# Autodesk Inventor assembly: 2AM-17-A-5200 - claw
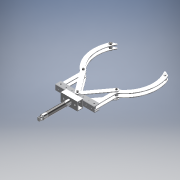
[picture p0: Inventor's stored thumbnail of the model, 180x180]
Saved by Autodesk Inventor 2017 (Build 210142000, 142)
## iProperties
Created: 2017-12-27
Part Number: 2AM-17-A-5200 - claw
Document SubType Name: Assembly
Designer: Micah
Mass: 406.083 g
Surface Area: 1172.05 cm^2
Volume: 145.474 cm^3
Density: 2.79145 g/cm^3
Author: Micah
## Documents named in this file (12)
- C:\Users\Micah\Desktop\inventor\CADathon-2017\2AM-17-A-0200 - Smokestack Elevator\2AM-17-A-5200 - claw.iam
- C:\Users\Micah\Desktop\inventor\CADathon-2017\2AM-17-A-0200 - Smokestack Elevator\2AM-17-A-6200 - claw arm.iam
- C:\Users\Micah\Desktop\inventor\CADathon-2017\2AM-17-A-0200 - Smokestack Elevator\2AM-17-P-5204 - links.ipt
- C:\Users\Micah\Desktop\inventor\CADathon-2017\2AM-17-A-0200 - Smokestack Elevator\2AM-17-P-5205 - c channel.ipt
- C:\Users\Micah\Desktop\inventor\CADathon-2017\2AM-17-A-0200 - Smokestack Elevator\2AM-17-P-5207 - supports spacer 09.ipt
- C:\Users\Micah\Desktop\inventor\CADathon-2017\2AM-17-A-0200 - Smokestack Elevator\2AM-17-P-5208 - supports spacer 215.ipt
- C:\Users\Micah\Desktop\inventor\CADathon-2017\2AM-17-A-0200 - Smokestack Elevator\2AM-17-P-5209 - cylinder mount.ipt
- C:\Users\Micah\Desktop\inventor\CADathon-2017\2AM-17-A-0200 - Smokestack Elevator\COTS\PARTserver02017093005073711525079192d056f\AIS2016\042-DP(F,D-166-3)(F,D-9).iam
- C:\Users\Micah\Documents\Inventor\Content Center Files\R2017\en-US\IS 2269\IS 2269 - M5 x 40.ipt
- C:\Users\Micah\Desktop\inventor\CADathon-2017\2AM-17-A-0200 - Smokestack Elevator\COTS\PARTserver02017093005073711525079192d056f\AIS2016\rod1.iam
- C:\Users\Micah\Documents\Inventor\Content Center Files\R2017\en-US\ISO 4762(2)\ISO 4762 - M5 x 45ISO.ipt
- C:\Users\Micah\Documents\Inventor\Content Center Files\R2017\en-US\ANSI B18.2.4.5M\ANSI B18.2.4.5M - M5 x 0.8.ipt
## Components (20 placed, 11 different names)
1. 2AM-17-A-6200 - claw arm:1 [sub-assembly] — Mate:9, Mate:11, Rotational:1, Rotational:4
2. 2AM-17-P-5204 - links:1 — Mate:3, Mate:13, Flush:1, Insert:1, Insert:5
3. 2AM-17-P-5204 - links:2 — Mate:4, Cylindrical:1, Mate:15, Flush:1, Mate:27
4. 2AM-17-P-5204 - links:4 — Mate:3, Cylindrical:2, Mate:14, Flush:2, Insert:2
5. 2AM-17-P-5205 - c channel:1 — Cylindrical:1, Cylindrical:2, Mate:9, Mate:10, Mate:11, Mate:16, Mate:17, Mate:18, Mate:19
6. 2AM-17-P-5204 - links:5 — Mate:4, Mate:12, Flush:2, Mate:23, Mate:25
7. 2AM-17-A-6200 - claw arm:2 [sub-assembly] — Mate:10, Mate:16, Rotational:2, Rotational:3
8. 2AM-17-P-5207 - supports spacer 09:1 — Mate:15, Rotational:2
9. 2AM-17-P-5207 - supports spacer 09:2 — Mate:14, Rotational:4
10. 2AM-17-P-5208 - supports spacer 215:1 — Mate:12, Rotational:1
11. 2AM-17-P-5208 - supports spacer 215:2 — Mate:13, Rotational:3
12. 2AM-17-P-5209 - cylinder mount:1 — Mate:17, Mate:18, Mate:19, Mate:20
13. 042-DP(F,D-166-3)(F,D-9):1 [sub-assembly] — Mate:20, Mate:21
14. rod1:1 [sub-assembly] — Mate:21
15. IS 2269 M5 x 40:1 — Insert:1, Mate:26
16. IS 2269 M5 x 40:2 — Insert:2, Mate:24
17. ISO 4762 M5 x 45:1 — Insert:5, Mate:22
18. Hex Jam Nut - Metric M5 x 0.8:1 — Mate:22, Mate:23
19. Hex Jam Nut - Metric M5 x 0.8:2 — Mate:24, Mate:25
20. Hex Jam Nut - Metric M5 x 0.8:3 — Mate:26, Mate:27
## Relationships (32: Mate 21, RevoluteJoint 4, Insert 3, CylindricalJoint 2, Flush 2)
- Mate:3: 2AM-17-P-5204 - links:1 ↔ 2AM-17-P-5204 - links:4
- Mate:4: 2AM-17-P-5204 - links:2 ↔ 2AM-17-P-5204 - links:5
- Cylindrical:1: 2AM-17-P-5204 - links:2 ↔ 2AM-17-P-5205 - c channel:1
- Cylindrical:2: 2AM-17-P-5204 - links:4 ↔ 2AM-17-P-5205 - c channel:1
- Mate:9: 2AM-17-A-6200 - claw arm:1 ↔ 2AM-17-P-5205 - c channel:1
- Mate:10: 2AM-17-P-5205 - c channel:1 ↔ 2AM-17-A-6200 - claw arm:2
- Mate:11: 2AM-17-A-6200 - claw arm:1 ↔ 2AM-17-P-5205 - c channel:1
- Mate:12: 2AM-17-P-5204 - links:5 ↔ 2AM-17-P-5208 - supports spacer 215:1
- Mate:13: 2AM-17-P-5204 - links:1 ↔ 2AM-17-P-5208 - supports spacer 215:2
- Mate:14: 2AM-17-P-5204 - links:4 ↔ 2AM-17-P-5207 - supports spacer 09:2
- Mate:15: 2AM-17-P-5204 - links:2 ↔ 2AM-17-P-5207 - supports spacer 09:1
- Mate:16: 2AM-17-P-5205 - c channel:1 ↔ 2AM-17-A-6200 - claw arm:2
- Rotational:1 [RevoluteJoint]: 2AM-17-A-6200 - claw arm:1 ↔ 2AM-17-P-5208 - supports spacer 215:1
- Rotational:2 [RevoluteJoint]: 2AM-17-A-6200 - claw arm:2 ↔ 2AM-17-P-5207 - supports spacer 09:1
- Rotational:3 [RevoluteJoint]: 2AM-17-A-6200 - claw arm:2 ↔ 2AM-17-P-5208 - supports spacer 215:2
- Rotational:4 [RevoluteJoint]: 2AM-17-A-6200 - claw arm:1 ↔ 2AM-17-P-5207 - supports spacer 09:2
- Flush:1: 2AM-17-P-5204 - links:1 ↔ 2AM-17-P-5204 - links:2
- Flush:2: 2AM-17-P-5204 - links:4 ↔ 2AM-17-P-5204 - links:5
- Mate:17: 2AM-17-P-5205 - c channel:1 ↔ 2AM-17-P-5209 - cylinder mount:1
- Mate:18: 2AM-17-P-5205 - c channel:1 ↔ 2AM-17-P-5209 - cylinder mount:1
- Mate:19: 2AM-17-P-5205 - c channel:1 ↔ 2AM-17-P-5209 - cylinder mount:1
- Mate:20: 2AM-17-P-5209 - cylinder mount:1 ↔ 042-DP(F,D-166-3)(F,D-9):1
- Mate:21: 042-DP(F,D-166-3)(F,D-9):1 ↔ rod1:1
- Insert:1: 2AM-17-P-5204 - links:1 ↔ IS 2269 M5 x 40:1
- Insert:2: 2AM-17-P-5204 - links:4 ↔ IS 2269 M5 x 40:2
- Insert:5: 2AM-17-P-5204 - links:1 ↔ ISO 4762 M5 x 45:1
- Mate:22: ISO 4762 M5 x 45:1 ↔ Hex Jam Nut - Metric M5 x 0.8:1
- Mate:23: 2AM-17-P-5204 - links:5 ↔ Hex Jam Nut - Metric M5 x 0.8:1
- Mate:24: IS 2269 M5 x 40:2 ↔ Hex Jam Nut - Metric M5 x 0.8:2
- Mate:25: 2AM-17-P-5204 - links:5 ↔ Hex Jam Nut - Metric M5 x 0.8:2
- Mate:26: IS 2269 M5 x 40:1 ↔ Hex Jam Nut - Metric M5 x 0.8:3
- Mate:27: 2AM-17-P-5204 - links:2 ↔ Hex Jam Nut - Metric M5 x 0.8:3
